# Autodesk Inventor assembly: rendering_zemax_assembly
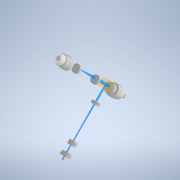
[picture p0: Inventor's stored thumbnail of the model, 180x180]
Saved by Autodesk Inventor 2021 (Build 250183000, 183)
## iProperties
Created: 2021-06-17
Part Number: rendering_zemax_assembly
Document SubType Name: Assembly
Designer: MicroscopyInnovation
Author: MicroscopyInnovation
## Documents named in this file (10)
- C:\Users\MicroscopyInnovation\Documents\Inventor\NatProtocolsManuscript\rendering_zemax_assembly.iam
- C:\Users\MicroscopyInnovation\Documents\Inventor\NatProtocolsManuscript\optics_54_10_12_multi_immersion_objective.ipt
- C:\Users\MicroscopyInnovation\Documents\Inventor\NatProtocolsManuscript\rendering_ACY254_050_A.ipt
- C:\Users\MicroscopyInnovation\Documents\Inventor\NatProtocolsManuscript\rendering_AC254_060_A.ipt
- C:\Users\MicroscopyInnovation\Documents\Inventor\NatProtocolsManuscript\rendering_AC254_040_A.ipt
- C:\Users\MicroscopyInnovation\Documents\Inventor\NatProtocolsManuscript\rendering_PBS251.ipt
- C:\Users\MicroscopyInnovation\Documents\Inventor\NatProtocolsManuscript\ASLM_100_40lensPair.ipt
- C:\Users\MicroscopyInnovation\Documents\Inventor\NatProtocolsManuscript\AQWP10M-580.ipt
- C:\Users\MicroscopyInnovation\Documents\Inventor\NatProtocolsManuscript\AHWP10M-580-Step.ipt
- C:\Users\MicroscopyInnovation\Documents\Inventor\NatProtocolsManuscript\PF05-03-G01.ipt
## Components (11 placed, 9 different names)
1. optics_54_10_12_multi_immersion_objective:1 — Angle:2, Mate:10, Mate:11, Mate:12, Mate:15
2. rendering_ACY254_050_A:1 — Mate:1, Angle:1, Mate:14
3. rendering_AC254_060_A:1 — Mate:4, Mate:15
4. rendering_AC254_060_A:2 — Mate:1, Angle:1
5. rendering_AC254_040_A:1 — Mate:4, Mate:12
6. rendering_PBS251:1 — Angle:2, Mate:10
7. optics_54_10_12_multi_immersion_objective:2 — Mate:11, Mate:13, Mate:16
8. ASLM_100_40lensPair:1
9. AQWP10M-580:1 — Mate:13
10. AHWP10M-580-Step:1 — Mate:14
11. PF05-03-G01:1 — Mate:16
## Relationships (11: Mate 9, Angle 2)
- Mate:1: rendering_ACY254_050_A:1 ↔ rendering_AC254_060_A:2
- Angle:1 (0 deg): rendering_ACY254_050_A:1 ↔ rendering_AC254_060_A:2
- Mate:4: rendering_AC254_060_A:1 ↔ rendering_AC254_040_A:1
- Angle:2 (0 deg): optics_54_10_12_multi_immersion_objective:1 ↔ rendering_PBS251:1
- Mate:10 (180 mm): optics_54_10_12_multi_immersion_objective:1 ↔ rendering_PBS251:1
- Mate:11: optics_54_10_12_multi_immersion_objective:1 ↔ optics_54_10_12_multi_immersion_objective:2
- Mate:12 (50 mm): optics_54_10_12_multi_immersion_objective:1 ↔ rendering_AC254_040_A:1
- Mate:13: optics_54_10_12_multi_immersion_objective:2 ↔ AQWP10M-580:1
- Mate:14: rendering_ACY254_050_A:1 ↔ AHWP10M-580-Step:1
- Mate:15: optics_54_10_12_multi_immersion_objective:1 ↔ rendering_AC254_060_A:1
- Mate:16: optics_54_10_12_multi_immersion_objective:2 ↔ PF05-03-G01:1
